# Autodesk Inventor assembly: Gripper
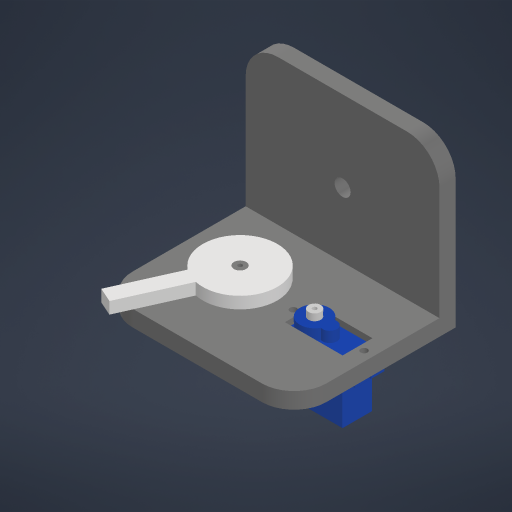
[picture p0: Inventor's stored thumbnail of the model, 512x512]
Saved by Autodesk Inventor 2023 (Build 270158000, 158)
## iProperties
Created: 2022-11-05
Part Number: Gripper
Document SubType Name: Assembly
Designer: cmzgt
Author: cmzgt
## Documents named in this file (4)
- D:\Projects\RoboArm\Gripper\Gripper.iam
- D:\Projects\RoboArm\Gripper\Base.ipt
- D:\Projects\RoboArm\Gripper\Servo.ipt
- D:\Projects\RoboArm\Gripper\Driver.ipt
## Components (3 placed, 3 different names)
1. Base:1 — Mate:1, Flush:1, Flush:2, Rotational:1
2. Servo:1 — Mate:1, Flush:1, Flush:2
3. Driver:1 — Rotational:1
## Relationships (4: Flush 2, Mate 1, RevoluteJoint 1)
- Mate:1: Base:1 ↔ Servo:1
- Flush:1 (25.4 mm): Base:1 ↔ Servo:1
- Flush:2 (6.35 mm): Base:1 ↔ Servo:1
- Rotational:1 [RevoluteJoint]: Base:1 ↔ Driver:1
